# Autodesk Inventor assembly: EnsamblePata
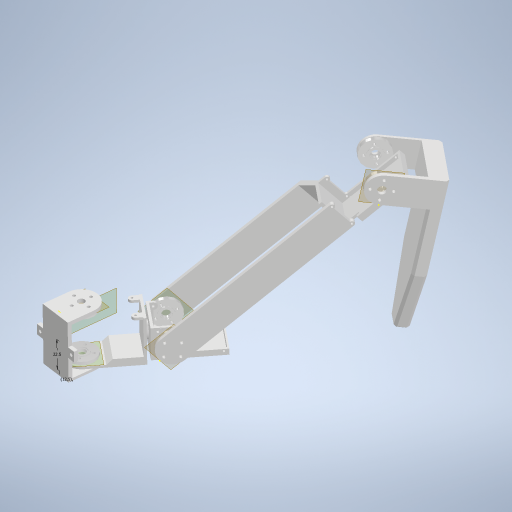
[picture p0: Inventor's stored thumbnail of the model, 512x512]
Saved by Autodesk Inventor 2024 (Build 280153000, 153)
## iProperties
Created: 2024-03-17
Part Number: EnsamblePata
Document SubType Name: Assembly
Designer: na_re
Author: na_re
## Documents named in this file (9)
- C:\Users\na_re\OneDrive\Escritorio\CAD_NAOMI\EnsamblePata.iam
- C:\Users\Public\Documents\Autodesk\Inventor 2024\HEXAPOD_CAD\YB-SD15M_LD v6_1.iam
- C:\Users\Public\Documents\Autodesk\Inventor 2024\HEXAPOD_CAD\RudderDisk v2.ipt
- C:\Users\Public\Documents\Autodesk\Inventor 2024\HEXAPOD_CAD\AuxRudderDisk v2.ipt
- C:\Users\Public\Documents\Autodesk\Inventor 2024\UnionCuerpo.ipt
- C:\Users\Public\Documents\Autodesk\Inventor 2024\HEXAPOD_CAD\Coxa.ipt
- C:\Users\Public\Documents\Autodesk\Inventor 2024\HEXAPOD_CAD\femurAux.ipt
- C:\Users\Public\Documents\Autodesk\Inventor 2024\HEXAPOD_CAD\tibiaMot.ipt
- C:\Users\Public\Documents\Autodesk\Inventor 2024\HEXAPOD_CAD\tibia.ipt
## Components (14 placed, 8 different names)
1. YB-SD15M_LD v6_1:1 [sub-assembly] — Coincidencia:2
2. RudderDisk v2:1 — De rotación:3
3. AuxRudderDisk v2:1 — De rotación:4
4. UnionCuerpo:1 — De rotación:3
5. Coxa:1 — De rotación:4, Coincidencia:2, De rotación:7, Coincidencia:4
6. YB-SD15M_LD v6_1:2 [sub-assembly] — De rotación:7, Coincidencia:4
7. RudderDisk v2:2 — De rotación:8
8. AuxRudderDisk v2:2 — De rotación:9
9. femurAux:1 — De rotación:9, Coincidencia:6, Coincidencia:7, Coincidencia:8
10. femurMot:1 — De rotación:8, Coincidencia:9
11. YB-SD15M_LD v6_1:3 [sub-assembly] — Coincidencia:6, Coincidencia:7, Coincidencia:8, Coincidencia:9
12. RudderDisk v2:3 — Nivelación:1, Nivelación:2, De rotación:12
13. AuxRudderDisk v2:3
14. tibia:1 — Nivelación:1, Nivelación:2, De rotación:12
## Relationships (23: RevoluteJoint 12, Mate 9, Flush 2)
- [RevoluteJoint]: YB-SD15M_LD v6_1:1 ↔ RudderDisk v2:1
- [Mate] (3.5 mm): YB-SD15M_LD v6_1:1 ↔ RudderDisk v2:1
- [RevoluteJoint] (1.4 mm): YB-SD15M_LD v6_1:1 ↔ AuxRudderDisk v2:1
- De rotación:3 [RevoluteJoint]: RudderDisk v2:1 ↔ UnionCuerpo:1
- De rotación:4 [RevoluteJoint]: AuxRudderDisk v2:1 ↔ Coxa:1
- Coincidencia:2 [Mate]: YB-SD15M_LD v6_1:1 ↔ Coxa:1
- [RevoluteJoint]: YB-SD15M_LD v6_1:2 ↔ RudderDisk v2:2
- [Mate] (3.5 mm): YB-SD15M_LD v6_1:2 ↔ RudderDisk v2:2
- [RevoluteJoint] (1.4 mm): YB-SD15M_LD v6_1:2 ↔ AuxRudderDisk v2:2
- De rotación:7 [RevoluteJoint]: Coxa:1 ↔ YB-SD15M_LD v6_1:2
- Coincidencia:4 [Mate]: Coxa:1 ↔ YB-SD15M_LD v6_1:2
- De rotación:8 [RevoluteJoint]: RudderDisk v2:2 ↔ femurMot:1
- De rotación:9 [RevoluteJoint]: AuxRudderDisk v2:2 ↔ femurAux:1
- [RevoluteJoint]: YB-SD15M_LD v6_1:3 ↔ RudderDisk v2:3
- [Mate] (3.5 mm): YB-SD15M_LD v6_1:3 ↔ RudderDisk v2:3
- [RevoluteJoint] (1.4 mm): YB-SD15M_LD v6_1:3 ↔ AuxRudderDisk v2:3
- Coincidencia:6 [Mate]: femurAux:1 ↔ YB-SD15M_LD v6_1:3
- Coincidencia:7 [Mate]: femurAux:1 ↔ YB-SD15M_LD v6_1:3
- Coincidencia:8 [Mate]: femurAux:1 ↔ YB-SD15M_LD v6_1:3
- Coincidencia:9 [Mate]: femurMot:1 ↔ YB-SD15M_LD v6_1:3
- Nivelación:1 [Flush]: RudderDisk v2:3 ↔ tibia:1
- Nivelación:2 [Flush]: RudderDisk v2:3 ↔ tibia:1
- De rotación:12 [RevoluteJoint]: RudderDisk v2:3 ↔ tibia:1
## Named parameters: d106_d87 = 0 mm, d107_d88 = -160.664515 deg, d108_d89 = 3.5 mm, d109_d96 = 1.4 mm, d110_d97 = 116.193544 deg, d125_d106_d87 = 0 mm, d126_d107_d88 = -37.065208 deg, d127_d108_d89 = 3.5 mm, d128_d109_d96 = 1.4 mm, d129_d110_d97 = 143.548906 deg
